# Autodesk Inventor assembly: Assembly_HCMUTE-CDT23_BE-TRUOT
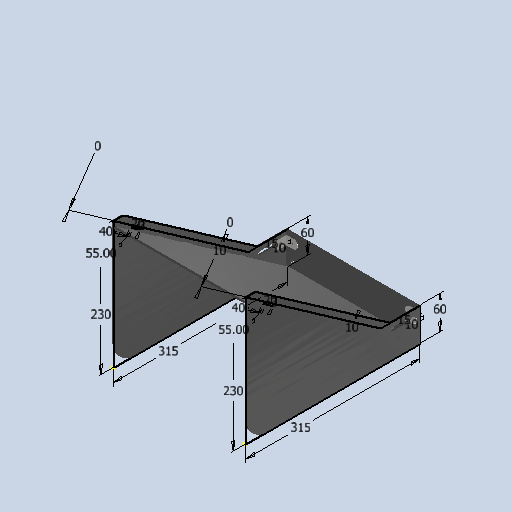
[picture p0: Inventor's stored thumbnail of the model, 512x512]
Saved by Autodesk Inventor 2023 (Build 270158000, 158)
## iProperties
Created: 2023-10-13
Part Number: Assembly_HCMUTE-CDT23_BE-TRUOT
Document SubType Name: Assembly
Designer: havie
Author: havie
## Documents named in this file (6)
- D:\DO_AN_CDT\1.1. PART\Part_Contain-Sample\Assembly_HCMUTE-CDT23_BE-TRUOT.iam
- D:\DO_AN_CDT\1.PART\Part_Contain-Sample\2309HCMUTE-CDT23_KE-GOC-20X20X16.ipt
- D:\DO_AN_CDT\1.PART\Part_Contain-Sample\2309HCMUTE-CDT23_TAM-GA.ipt
- D:\DO_AN_CDT\1.PART\Part_Contain-Sample\2309HCMUTE-CDT23_VACH-NGAN.ipt
- D:\DO_AN_CDT\1.PART\Part_Contain-Sample\2309HCMUTE-CDT23-MAT_TRUOT.ipt
- C:\Users\havie\Documents\Inventor\Content Center Files\R2023\en-US\ISO 4762(2)\ISO 4762 - M5 x 8ISO.ipt
## Components (8 placed, 5 different names)
1. 2309HCMUTE-CDT23_TAM-GA:1 — Mate:3, Mate:4, Angle:2, Mate:11, Mate:12, Angle:3, Flush:1
2. 2309HCMUTE-CDT23_VACH-NGAN:1 — Mate:6, Mate:7, Mate:15, Mate:16
3. 2309HCMUTE-CDT23_KE-GOC-20X20X16:2 — Mate:3, Mate:4, Angle:2, Mate:6, Mate:7
4. 2309HCMUTE-CDT23_VACH-NGAN:2 — Mate:13, Mate:14, Flush:1, Mate:17, Mate:18, Mate:19, Mate:20, Flush:2
5. 2309HCMUTE-CDT23_KE-GOC-20X20X16:4 — Mate:11, Mate:12, Mate:13, Mate:14, Angle:3
6. ISO 4762 M5 x 8:1 — Mate:17, Mate:18
7. ISO 4762 M5 x 8:2 — Mate:15, Mate:16
8. 2309HCMUTE-CDT23-MAT_TRUOT:1 — Mate:19, Mate:20, Flush:2
## Relationships (18: Mate 14, Angle 2, Flush 2)
- Mate:3: 2309HCMUTE-CDT23_TAM-GA:1 ↔ 2309HCMUTE-CDT23_KE-GOC-20X20X16:2
- Mate:4: 2309HCMUTE-CDT23_TAM-GA:1 ↔ 2309HCMUTE-CDT23_KE-GOC-20X20X16:2
- Angle:2 (0 deg): 2309HCMUTE-CDT23_TAM-GA:1 ↔ 2309HCMUTE-CDT23_KE-GOC-20X20X16:2
- Mate:6: 2309HCMUTE-CDT23_VACH-NGAN:1 ↔ 2309HCMUTE-CDT23_KE-GOC-20X20X16:2
- Mate:7: 2309HCMUTE-CDT23_VACH-NGAN:1 ↔ 2309HCMUTE-CDT23_KE-GOC-20X20X16:2
- Mate:11: 2309HCMUTE-CDT23_TAM-GA:1 ↔ 2309HCMUTE-CDT23_KE-GOC-20X20X16:4
- Mate:12: 2309HCMUTE-CDT23_TAM-GA:1 ↔ 2309HCMUTE-CDT23_KE-GOC-20X20X16:4
- Mate:13: 2309HCMUTE-CDT23_VACH-NGAN:2 ↔ 2309HCMUTE-CDT23_KE-GOC-20X20X16:4
- Mate:14: 2309HCMUTE-CDT23_VACH-NGAN:2 ↔ 2309HCMUTE-CDT23_KE-GOC-20X20X16:4
- Angle:3 (0 deg): 2309HCMUTE-CDT23_TAM-GA:1 ↔ 2309HCMUTE-CDT23_KE-GOC-20X20X16:4
- Flush:1: 2309HCMUTE-CDT23_TAM-GA:1 ↔ 2309HCMUTE-CDT23_VACH-NGAN:2
- Mate:15: 2309HCMUTE-CDT23_VACH-NGAN:1 ↔ ISO 4762 M5 x 8:2
- Mate:16: 2309HCMUTE-CDT23_VACH-NGAN:1 ↔ ISO 4762 M5 x 8:2
- Mate:17: 2309HCMUTE-CDT23_VACH-NGAN:2 ↔ ISO 4762 M5 x 8:1
- Mate:18: 2309HCMUTE-CDT23_VACH-NGAN:2 ↔ ISO 4762 M5 x 8:1
- Mate:19: 2309HCMUTE-CDT23_VACH-NGAN:2 ↔ 2309HCMUTE-CDT23-MAT_TRUOT:1
- Mate:20: 2309HCMUTE-CDT23_VACH-NGAN:2 ↔ 2309HCMUTE-CDT23-MAT_TRUOT:1
- Flush:2: 2309HCMUTE-CDT23_VACH-NGAN:2 ↔ 2309HCMUTE-CDT23-MAT_TRUOT:1
